# Autodesk Inventor assembly: FullBot
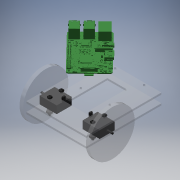
[picture p0: Inventor's stored thumbnail of the model, 180x180]
Saved by Autodesk Inventor 2018.1 (Build 221171000, 171)
## iProperties
Created: 2018-05-04
Part Number: FullBot
Document SubType Name: Assembly
Designer: mmarkle
Author: mmarkle
## Documents named in this file (7)
- C:\Users\mmarkle\Documents\Robotics\PiBots2018\FullBot.iam
- C:\Users\mmarkle\Documents\Robotics\PiBots2018\pibot_baseplate.ipt
- C:\Users\mmarkle\Documents\Robotics\PiBots2018\MotorWithEnclosure.ipt
- C:\Users\mmarkle\Documents\Robotics\PiBots2018\pibot_baseplate_battery.ipt
- C:\Users\mmarkle\Documents\Robotics\PiBots2018\Raspberry Pi 3_Shrinkwrap_1.ipt
- C:\Users\mmarkle\Documents\Robotics\PiBots2018\FullBot\Design Accelerator\Bolted Connection1.iam
- C:\Users\mmarkle\Documents\Robotics\PiBots2018\pibot_wheel_1.ipt
## Components (8 placed, 6 different names)
1. pibot_baseplate:1 — Mate:1, Mate:2, Mate:3, Mate:4, Mate:5, Mate:6
2. MotorWithEnclosure:1 — Mate:2, Mate:3, Mate:6, Mate:8, Mate:16, Angle:1, Flush:1
3. MotorWithEnclosure:2 — Mate:1, Mate:4, Mate:5, Mate:7, Mate:9, Mate:17, Angle:2, Flush:2
4. pibot_baseplate_battery:1 — Mate:7, Mate:8, Mate:9, Mate:12, Mate:13, Mate:14, Mate:15
5. Raspberry Pi 3_Shrinkwrap_1:1 — Mate:12, Mate:13
6. Bolted Connection:1 [sub-assembly] — Mate:14, Mate:15
7. pibot_wheel_1:1 — Mate:16, Angle:1, Flush:1
8. pibot_wheel_1:2 — Mate:17, Angle:2, Flush:2
## Relationships (19: Mate 15, Angle 2, Flush 2)
- Mate:1: pibot_baseplate:1 ↔ MotorWithEnclosure:2
- Mate:2: pibot_baseplate:1 ↔ MotorWithEnclosure:1
- Mate:3: pibot_baseplate:1 ↔ MotorWithEnclosure:1
- Mate:4: pibot_baseplate:1 ↔ MotorWithEnclosure:2
- Mate:5: pibot_baseplate:1 ↔ MotorWithEnclosure:2
- Mate:6: pibot_baseplate:1 ↔ MotorWithEnclosure:1
- Mate:7: MotorWithEnclosure:2 ↔ pibot_baseplate_battery:1
- Mate:8: MotorWithEnclosure:1 ↔ pibot_baseplate_battery:1
- Mate:9: MotorWithEnclosure:2 ↔ pibot_baseplate_battery:1
- Mate:12: pibot_baseplate_battery:1 ↔ Raspberry Pi 3_Shrinkwrap_1:1
- Mate:13: pibot_baseplate_battery:1 ↔ Raspberry Pi 3_Shrinkwrap_1:1
- Mate:14: pibot_baseplate_battery:1 ↔ Bolted Connection:1
- Mate:15: pibot_baseplate_battery:1 ↔ Bolted Connection:1
- Mate:16: MotorWithEnclosure:1 ↔ pibot_wheel_1:1
- Angle:1 (0 deg): MotorWithEnclosure:1 ↔ pibot_wheel_1:1
- Flush:1 (-1.27 mm): MotorWithEnclosure:1 ↔ pibot_wheel_1:1
- Mate:17: MotorWithEnclosure:2 ↔ pibot_wheel_1:2
- Angle:2 (0 deg): MotorWithEnclosure:2 ↔ pibot_wheel_1:2
- Flush:2 (1.27 mm): MotorWithEnclosure:2 ↔ pibot_wheel_1:2
